# Autodesk Inventor assembly: claw
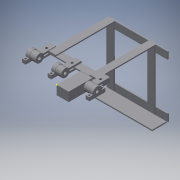
[picture p0: Inventor's stored thumbnail of the model, 180x180]
Saved by Autodesk Inventor 2017 (Build 210142000, 142)
## iProperties
Created: 2017-04-28
Part Number: claw
Document SubType Name: Assembly
Designer: s4321966
Author: s4321966
## Documents named in this file (5)
- \\puffball.labs.eait.uq.edu.au\s4321966\Documents\metr4810_spool draft\claw.iam
- \\puffball.labs.eait.uq.edu.au\s4321966\Documents\metr4810_spool draft\attachment.ipt
- \\puffball.labs.eait.uq.edu.au\s4321966\Documents\metr4810_spool draft\bar.ipt
- \\puffball.labs.eait.uq.edu.au\s4321966\Documents\metr4810_spool draft\servo attachment.ipt
- \\puffball.labs.eait.uq.edu.au\s4321966\Documents\metr4810_spool draft\servo.ipt
## Components (16 placed, 4 different names)
1. attachment:1 — Mate:9, Tangent:3, Flush:8
2. bar:1 — Flush:2, Mate:2, Flush:3, Flush:4, Flush:5, Mate:3, Flush:6, Mate:8, Mate:11, Flush:11, Flush:12, Mate:12
3. servo attachment:1 — Mate:1, Tangent:1, Flush:2, Mate:2, Flush:3, Mate:5, Tangent:4, Mate:10
4. servo:1 — Mate:1, Tangent:1, Flush:7, Flush:8, Flush:9, Flush:10
5. attachment:2 — Mate:5, Tangent:4, Flush:7, Flush:10
6. attachment:3 — Mate:4, Tangent:2, Flush:9
7. servo attachment:2 — Flush:4, Flush:5, Mate:3, Mate:4, Tangent:2, Mate:13
8. bar:2 — Mate:10, Mate:11, Flush:11, Flush:14, Mate:14, Flush:16
9. bar:3 — Flush:13, Flush:14, Flush:15, Mate:15, Flush:19
10. bar:4 — Flush:12, Mate:12, Mate:13, Flush:13, Flush:15, Flush:17, Mate:16
11. bar:5 — Mate:14, Mate:15, Flush:16, Flush:18, Mate:17
12. bar:6 — Flush:17, Mate:16, Flush:18, Flush:20, Mate:19, Flush:23, Flush:24
13. servo attachment:3 — Flush:6, Mate:8, Mate:9, Tangent:3
14. bar:7 — Mate:17, Flush:19, Flush:20
15. bar:8 — Mate:18, Flush:21, Flush:22
16. bar:9 — Mate:18, Flush:21, Flush:22, Mate:19, Flush:23, Flush:24
## Relationships (44: Flush 23, Mate 17, Tangent 4)
- Mate:1: servo attachment:1 ↔ servo:1
- Tangent:1: servo attachment:1 ↔ servo:1
- Flush:2: bar:1 ↔ servo attachment:1
- Mate:2: bar:1 ↔ servo attachment:1
- Flush:3: bar:1 ↔ servo attachment:1
- Flush:4: bar:1 ↔ servo attachment:2
- Flush:5: bar:1 ↔ servo attachment:2
- Mate:3: bar:1 ↔ servo attachment:2
- Mate:4: attachment:3 ↔ servo attachment:2
- Mate:5: servo attachment:1 ↔ attachment:2
- Flush:6: bar:1 ↔ servo attachment:3
- Mate:8: bar:1 ↔ servo attachment:3
- Mate:9: attachment:1 ↔ servo attachment:3
- Tangent:2: attachment:3 ↔ servo attachment:2
- Tangent:3: attachment:1 ↔ servo attachment:3
- Tangent:4: servo attachment:1 ↔ attachment:2
- Flush:7: servo:1 ↔ attachment:2
- Flush:8: attachment:1 ↔ servo:1
- Flush:9: servo:1 ↔ attachment:3
- Flush:10: servo:1 ↔ attachment:2
- Mate:10: servo attachment:1 ↔ bar:2
- Mate:11: bar:1 ↔ bar:2
- Flush:11: bar:1 ↔ bar:2
- Flush:12: bar:1 ↔ bar:4
- Mate:12: bar:1 ↔ bar:4
- Mate:13: servo attachment:2 ↔ bar:4
- Flush:13: bar:3 ↔ bar:4
- Flush:14: bar:2 ↔ bar:3
- Flush:15: bar:3 ↔ bar:4
- Mate:14: bar:2 ↔ bar:5
- Mate:15: bar:3 ↔ bar:5
- Flush:16: bar:2 ↔ bar:5
- Flush:17: bar:4 ↔ bar:6
- Mate:16: bar:4 ↔ bar:6
- Flush:18: bar:5 ↔ bar:6
- Mate:17: bar:5 ↔ bar:7
- Flush:19: bar:3 ↔ bar:7
- Flush:20: bar:6 ↔ bar:7
- Mate:18: bar:8 ↔ bar:9
- Flush:21: bar:8 ↔ bar:9
- Flush:22: bar:8 ↔ bar:9
- Mate:19: bar:6 ↔ bar:9
- Flush:23: bar:6 ↔ bar:9
- Flush:24: bar:6 ↔ bar:9
